# Autodesk Inventor assembly: ShooterAssemblyV06
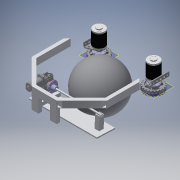
[picture p0: Inventor's stored thumbnail of the model, 180x180]
Saved by Autodesk Inventor 2016 SP1 (Build 200210100, 210)
## iProperties
Created: 2016-02-07
Part Number: ShooterAssemblyV06
Document SubType Name: Assembly
Designer: steele
Author: steele
## Documents named in this file (10)
- C:\snobotics\CAD-Development\robSteele\SnoBotics2016\2016-05-05-ShooterPrototype\ShooterAssemblyV06.iam
- C:\snobotics\CAD-Development\robSteele\SnoBotics2016\DraftOfBoulder.ipt
- C:\snobotics\CAD-Development\robSteele\SnoBotics2016\2016-05-05-ShooterPrototype\Mini_CIM_MotorHub_4_inch_wheel.iam
- C:\snobotics\CAD-Development\robSteele\SnoBotics2016\2016-05-05-ShooterPrototype\AluminumRodForShooter.ipt
- C:\snobotics\CAD-Development\robSteele\SnoBotics2016\AM Parts\am-0077a-500 Key Hub r2.ipt
- C:\snobotics\CAD-Development\robSteele\SnoBotics2016\AM Parts\SnowBlowerMotorAndHub.iam
- C:\snobotics\CAD-Development\robSteele\SnoBotics2016\AM Parts\rsSnowBlowerMount.ipt
- C:\snobotics\CAD-Development\robSteele\SnoBotics2016\2016-05-05-ShooterPrototype\SupportPlateToAttachToRobotBase.ipt
- C:\snobotics\CAD-Development\robSteele\SnoBotics2016\2016-05-05-ShooterPrototype\CIM_MotorHub_4_inch_wheel.iam
- C:\snobotics\CAD-Development\robSteele\SnoBotics2016\2016-05-05-ShooterPrototype\ShooterFrameAssembly05.iam
## Components (9 placed, 9 different names)
1. ShooterFrameAssembly05:1 [sub-assembly]
2. Mini_CIM_MotorHub_4_inch_wheel:1 [sub-assembly] — Mate:3, Mate:9, Flush:5
3. DraftOfBoulder:1 — Mate:3
4. AluminumRodForShooter:1 — Mate:9, Mate:10, Insert:1, Insert:4
5. am-0077a-500 Key Hub r2:1 — Insert:1, Insert:2
6. SnowBlowerMotorAndHub:1 [sub-assembly] — Insert:2, Insert:3
7. CIM_MotorHub_4_inch_wheel:1 [sub-assembly] — Flush:5
8. rsSnowBlowerMount:1 — Insert:3, Mate:13
9. SupportPlateToAttachToRobotBase:1 — Insert:4, Mate:13
## Relationships (17: Mate 10, Insert 4, Flush 3)
- [Mate]: ShooterFrameAssembly05:1 ↔ Mini_CIM_MotorHub_4_inch_wheel:1
- [Flush]: ShooterFrameAssembly05:1 ↔ Mini_CIM_MotorHub_4_inch_wheel:1
- [Flush] (-4.7625 mm): ShooterFrameAssembly05:1 ↔ Mini_CIM_MotorHub_4_inch_wheel:1
- [Mate]: ShooterFrameAssembly05:1 ↔ DraftOfBoulder:1
- Mate:3: Mini_CIM_MotorHub_4_inch_wheel:1 ↔ DraftOfBoulder:1
- [Mate]: ShooterFrameAssembly05:1 ↔ DraftOfBoulder:1
- Mate:9: Mini_CIM_MotorHub_4_inch_wheel:1 ↔ AluminumRodForShooter:1
- Mate:10: AluminumRodForShooter:1
- [Mate]: ShooterFrameAssembly05:1 ↔ AluminumRodForShooter:1
- Insert:1: AluminumRodForShooter:1 ↔ am-0077a-500 Key Hub r2:1
- Insert:2: am-0077a-500 Key Hub r2:1 ↔ SnowBlowerMotorAndHub:1
- Insert:3: SnowBlowerMotorAndHub:1 ↔ rsSnowBlowerMount:1
- Insert:4: AluminumRodForShooter:1 ↔ SupportPlateToAttachToRobotBase:1
- Mate:13: rsSnowBlowerMount:1 ↔ SupportPlateToAttachToRobotBase:1
- [Mate]: ShooterFrameAssembly05:1 ↔ CIM_MotorHub_4_inch_wheel:1
- [Mate]: ShooterFrameAssembly05:1 ↔ CIM_MotorHub_4_inch_wheel:1
- Flush:5: Mini_CIM_MotorHub_4_inch_wheel:1 ↔ CIM_MotorHub_4_inch_wheel:1
